# Autodesk Inventor assembly: AssemblyCFD
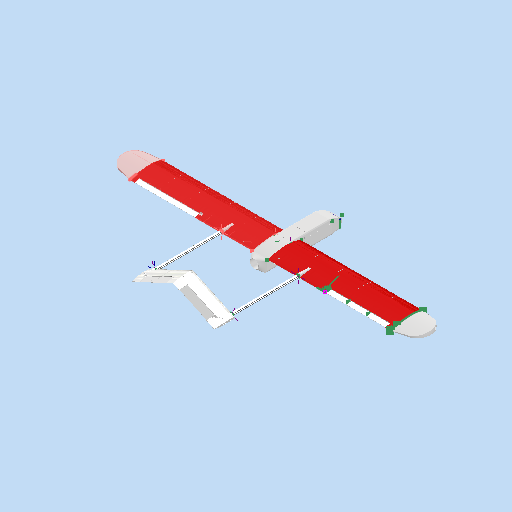
[picture p0: Inventor's stored thumbnail of the model, 512x512]
Saved by Autodesk Inventor 2026.1 (Build 301233000, 233)
## iProperties
Created: 2026-03-19
Part Number: AssemblyCFD
Document SubType Name: Assembly
Designer: mateo
Author: mateo
## Documents named in this file (11)
- C:\GitHub\Senior-Design-UAV\Elytra CAD\CFD Assembly\AssemblyCFD.iam
- C:\GitHub\Senior-Design-UAV\Elytra CAD\CFD Parts\Fueselage.ipt
- C:\GitHub\Senior-Design-UAV\Elytra CAD\20x20 Extrusions\20x20x2900ExtrudedAluminum.ipt
- C:\GitHub\Senior-Design-UAV\Elytra CAD\CFD Parts\WingLeftCFD.ipt
- C:\GitHub\Senior-Design-UAV\Elytra CAD\CFD Parts\WingMirrorCFD.ipt
- C:\GitHub\Senior-Design-UAV\Elytra CAD\CFD Assembly\TailCFDAssembly.iam
- C:\GitHub\Senior-Design-UAV\Elytra CAD\20x20 Extrusions\20x20x800ExtrudedAluminum.ipt
- C:\GitHub\Senior-Design-UAV\Elytra CAD\CFD Parts\Cover2.ipt
- C:\GitHub\Senior-Design-UAV\Elytra CAD\CFD Parts\AlerionLeft.ipt
- C:\GitHub\Senior-Design-UAV\Elytra CAD\CFD Parts\AlerionLeft_MIR.ipt
- C:\GitHub\Senior-Design-UAV\Elytra CAD\Landing Gear\LandingGearNose2.iam
## Components (13 placed, 10 different names)
1. Fueselage:1 — Mate:1, Mate:2, Mate:5, Mate:6, Mate:9, Mate:10, Mate:17
2. 20x20x2900ExtrudedAluminum:1 — Mate:5, Mate:6, Mate:7, Mate:8, Mate:13, Mate:14
3. WingLeftCFD:1 — Mate:7, Mate:9, Mate:11, Insert:1
4. WingMirrorCFD:1 — Mate:8, Mate:10, Mate:12
5. TailCFDAssembly:1 [sub-assembly] — Mate:15, Mate:16
6. 20x20x800ExtrudedAluminum:1 — Mate:11, Mate:14, Mate:15, Mate:16
7. 20x20x800ExtrudedAluminum:2 — Mate:12, Mate:13
8. Cover2:1 — Mate:17
9. AlerionLeft:1 — Insert:1
10. AlerionLeft_MIR:1
11. LandingGearNose2:1 [sub-assembly]
12. LandingGearNose2:2 [sub-assembly]
13. LandingGearNose2:3 [sub-assembly]
## Relationships (16: Mate 15, Insert 1)
- Mate:1: Fueselage:1
- Mate:2: Fueselage:1
- Mate:5: Fueselage:1 ↔ 20x20x2900ExtrudedAluminum:1
- Mate:6: Fueselage:1 ↔ 20x20x2900ExtrudedAluminum:1
- Mate:7: 20x20x2900ExtrudedAluminum:1 ↔ WingLeftCFD:1
- Mate:8: 20x20x2900ExtrudedAluminum:1 ↔ WingMirrorCFD:1
- Mate:9: Fueselage:1 ↔ WingLeftCFD:1
- Mate:10: Fueselage:1 ↔ WingMirrorCFD:1
- Mate:11: WingLeftCFD:1 ↔ 20x20x800ExtrudedAluminum:1
- Mate:12: WingMirrorCFD:1 ↔ 20x20x800ExtrudedAluminum:2
- Mate:13: 20x20x2900ExtrudedAluminum:1 ↔ 20x20x800ExtrudedAluminum:2
- Mate:14: 20x20x2900ExtrudedAluminum:1 ↔ 20x20x800ExtrudedAluminum:1
- Mate:15: TailCFDAssembly:1 ↔ 20x20x800ExtrudedAluminum:1
- Mate:16 (-3 mm): TailCFDAssembly:1 ↔ 20x20x800ExtrudedAluminum:1
- Mate:17: Fueselage:1 ↔ Cover2:1
- Insert:1: WingLeftCFD:1 ↔ AlerionLeft:1
